# Autodesk Inventor assembly: racked
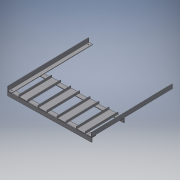
[picture p0: Inventor's stored thumbnail of the model, 180x180]
Saved by Autodesk Inventor 2017 (Build 210142000, 142)
## iProperties
Created: 2018-10-17
Part Number: racked
Document SubType Name: Assembly
Designer: ddeboer
Author: ddeboer
## Documents named in this file (3)
- C:\Users\ddeboer\Desktop\snap_holder\racked.iam
- C:\Users\ddeboer\Desktop\snap_holder\channel.ipt
- C:\Users\ddeboer\Desktop\snap_holder\uchannel.ipt
## Components (8 placed, 2 different names)
1. channel:1 — Insert:2, Flush:4, Mate:2, Flush:5, Mate:3, Insert:3, Flush:6
2. channel:2 — Mate:1, Flush:3, Mate:2
3. channel:3 — Insert:2, Mate:1, Flush:3, Flush:4, Mate:4
4. channel:4 — Insert:3, Flush:6
5. uchannel:1 — Flush:5, Mate:3, Mate:4
6. uchannel:2
7. uchannel:3
8. uchannel:4
## Component patterns: (4 elements, first: uchannel:1)
## Relationships (10: Mate 4, Flush 4, Insert 2)
- Insert:2: channel:1 ↔ channel:3
- Mate:1: channel:2 ↔ channel:3
- Flush:3: channel:2 ↔ channel:3
- Flush:4: channel:1 ↔ channel:3
- Mate:2 (152.4 mm): channel:1 ↔ channel:2
- Flush:5: channel:1 ↔ uchannel:1
- Mate:3: channel:1 ↔ uchannel:1
- Mate:4 (63.5 mm): channel:3 ↔ uchannel:1
- Insert:3: channel:1 ↔ channel:4
- Flush:6: channel:1 ↔ channel:4
